# Autodesk Inventor assembly: ZAxisRodClamp
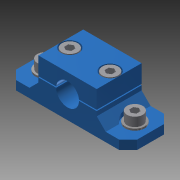
[picture p0: Inventor's stored thumbnail of the model, 180x180]
Saved by Autodesk Inventor 2015 SP1 (Build 190203100, 203)
## iProperties
Created: 2015-01-29
Part Number: ZAxisRodClamp
Document SubType Name: Assembly
Designer: Jack
Mass: 12.8501 g
Surface Area: 75.7343 cm^2
Volume: 10.4635 cm^3
Density: 1.22809 g/cm^3
Author: Jack
Title: Z Axis Rod Clamp
## Documents named in this file (6)
- C:\Users\Jack\ownCloud\Projects\CrossBot\InventorModel\ZAxis\ZAxisRodClamp.iam
- C:\Users\Jack\ownCloud\Projects\CrossBot\InventorModel\ZAxis\ZAxisRodClampBody.ipt
- C:\Users\Jack\ownCloud\Projects\CrossBot\InventorModel\ZAxis\ZAxisRodClampTop.ipt
- C:\Users\Jack\ownCloud\Projects\CrossBot\InventorModel\Hardware\BoltWashers\BoltWasher4\BoltWasher4x10.iam
- C:\Users\Jack\ownCloud\Projects\CrossBot\InventorModel\Hardware\Bolts\SHCS\SHCS4\SHCS4x14.ipt
- C:\Users\Jack\ownCloud\Projects\CrossBot\InventorModel\Hardware\Nuts\Nut4.ipt
## Components (8 placed, 5 different names)
1. ZAxisRodClampBody:1 — Mate:4, Mate:5, Mate:6, Mate:7, Mate:14, Mate:15, Angle:1, Angle:2
2. ZAxisRodClampTop:1 — Mate:8, Mate:9, Mate:10, Mate:11
3. BoltWasher4x10:1 [sub-assembly] — Mate:5, Mate:6
4. BoltWasher4x10:2 [sub-assembly] — Mate:4, Mate:7
5. SHCS4x14:1 — Mate:8, Mate:11, Mate:13
6. SHCS4x14:2 — Mate:9, Mate:10, Mate:12
7. Nut4:1 — Mate:13, Mate:14, Angle:2
8. Nut4:2 — Mate:12, Mate:15, Angle:1
## Relationships (17: Mate 15, Angle 2)
- [Mate]: ZAxisRodClampBody:1 ↔ ZAxisRodClampTop:1
- [Mate]: ZAxisRodClampBody:1 ↔ ZAxisRodClampTop:1
- [Mate] (0.5 mm): ZAxisRodClampBody:1 ↔ ZAxisRodClampTop:1
- Mate:4: ZAxisRodClampBody:1 ↔ BoltWasher4x10:2
- Mate:5: ZAxisRodClampBody:1 ↔ BoltWasher4x10:1
- Mate:6: ZAxisRodClampBody:1 ↔ BoltWasher4x10:1
- Mate:7: ZAxisRodClampBody:1 ↔ BoltWasher4x10:2
- Mate:8: ZAxisRodClampTop:1 ↔ SHCS4x14:1
- Mate:9: ZAxisRodClampTop:1 ↔ SHCS4x14:2
- Mate:10: ZAxisRodClampTop:1 ↔ SHCS4x14:2
- Mate:11: ZAxisRodClampTop:1 ↔ SHCS4x14:1
- Mate:12: SHCS4x14:2 ↔ Nut4:2
- Mate:13: SHCS4x14:1 ↔ Nut4:1
- Mate:14: ZAxisRodClampBody:1 ↔ Nut4:1
- Mate:15: ZAxisRodClampBody:1 ↔ Nut4:2
- Angle:1 (0 deg): ZAxisRodClampBody:1 ↔ Nut4:2
- Angle:2 (0 deg): ZAxisRodClampBody:1 ↔ Nut4:1
## Named parameters: d271_d261 = 0 mm, d272_d262 = 0 mm, d273_d263 = 0.5 mm
